# Autodesk Inventor assembly: ElectricCore
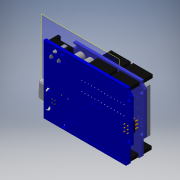
[picture p0: Inventor's stored thumbnail of the model, 180x180]
Saved by Autodesk Inventor 2016 (Build 200138000, 138)
## iProperties
Created: 2017-06-15
Part Number: ElectricCore
Document SubType Name: Assembly
Designer: Owner
Author: Owner
## Documents named in this file (4)
- C:\Users\Owner\Documents\Inventor\TSA\2017\Animatronics\Alligator\Mock Parts\ElectricCore.iam
- C:\Users\Owner\Documents\Inventor\TSA\2017\Animatronics\Alligator\Mock Parts\arduino-uno.snapshot.3\arduino uno.iam
- C:\Users\Owner\Documents\Inventor\TSA\2017\Animatronics\Alligator\Mock Parts\Protoshield\arduino uno.iam
- C:\Users\Owner\Documents\Inventor\TSA\2017\Animatronics\Alligator\Mock Parts\Breadboard.ipt
## Components (3 placed, 2 different names)
1. arduino uno:1 [sub-assembly] — Mate:1, Flush:1, Flush:2
2. arduino uno:2 [sub-assembly] — Mate:1, Flush:1, Flush:2, Flush:3, Flush:4
3. Breadboard:1 — Flush:3, Flush:4
## Relationships (5: Flush 4, Mate 1)
- Mate:1: arduino uno:1 ↔ arduino uno:2
- Flush:1: arduino uno:1 ↔ arduino uno:2
- Flush:2: arduino uno:1 ↔ arduino uno:2
- Flush:3: arduino uno:2 ↔ Breadboard:1
- Flush:4: arduino uno:2 ↔ Breadboard:1
